# Autodesk Inventor assembly: X-axis Assembly
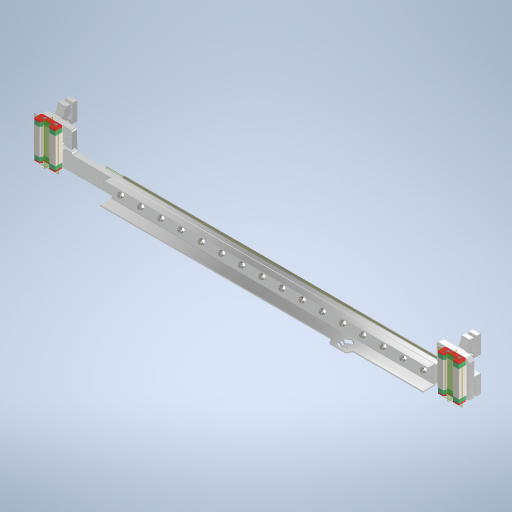
[picture p0: Inventor's stored thumbnail of the model, 512x512]
Saved by Autodesk Inventor 2024 (Build 280153000, 153)
## iProperties
Created: 2024-08-04
Part Number: X-axis Assembly
Document SubType Name: Assembly
Designer: Ishaan
Author: Ishaan
## Documents named in this file (9)
- E:\Projects\Axiom--IDEX-3D-Printer\CAD\12 - X-axis\X-axis Assembly.iam
- E:\Projects\Axiom--IDEX-3D-Printer\CAD\00 - COTS Components\MGN12H\MGN12H, LINEAR GUIDE BLOCK.ipt
- E:\Projects\Axiom--IDEX-3D-Printer\CAD\00 - COTS Components\MGNR12 400mm Rail\MGNR12R400HM.ipt
- E:\Projects\Axiom--IDEX-3D-Printer\CAD\12 - X-axis\Gantry Belt Clamp.ipt
- E:\Projects\Axiom--IDEX-3D-Printer\CAD\12 - X-axis\Gantry Stiffener.ipt
- E:\Projects\Axiom--IDEX-3D-Printer\CAD\00 - COTS Components\Hardware\SHCSM3x8.ipt
- E:\Projects\Axiom--IDEX-3D-Printer\CAD\00 - COTS Components\Hardware\SHCSM3x16.ipt
- E:\Projects\Axiom--IDEX-3D-Printer\CAD\00 - COTS Components\Hardware\M3 LOCKNUT.ipt
- E:\Projects\Axiom--IDEX-3D-Printer\CAD\12 - X-axis\R3 Gantry Bar.ipt
## Components (51 placed, 8 different names)
1. MGN12H, LINEAR GUIDE BLOCK:1
2. MGN12H, LINEAR GUIDE BLOCK:2
3. MGNR12R400HM:1 — Insert:121
4. R3 Gantry Bar:1
5. Gantry Belt Clamp:1 — Insert:119, Insert:120
6. Gantry Belt Clamp:2 — Insert:117, Insert:118
7. Gantry Stiffener:1 — Insert:122
8. SHCSM3x8:1
9. SHCSM3x8:2
10. SHCSM3x8:3
11. SHCSM3x8:4
12. SHCSM3x8:5
13. SHCSM3x8:6
14. SHCSM3x8:7
15. SHCSM3x8:8
16. SHCSM3x16:1 — Insert:117
17. SHCSM3x16:2 — Insert:118
18. SHCSM3x16:3 — Insert:119
19. SHCSM3x16:4 — Insert:120
20. SHCSM3x16:5 — Insert:121
21. SHCSM3x16:6
22. SHCSM3x16:7
23. SHCSM3x16:8
24. SHCSM3x16:9
25. SHCSM3x16:10
26. SHCSM3x16:11
27. SHCSM3x16:12
28. SHCSM3x16:13
29. SHCSM3x16:14
30. SHCSM3x16:15
31. SHCSM3x16:16
32. SHCSM3x16:17
33. SHCSM3x16:18
34. SHCSM3x16:19
35. SHCSM3x16:20
36. M3 LOCKNUT:1 — Insert:122
37. M3 LOCKNUT:2
38. M3 LOCKNUT:3
39. M3 LOCKNUT:4
40. M3 LOCKNUT:5
41. M3 LOCKNUT:6
42. M3 LOCKNUT:7
43. M3 LOCKNUT:8
44. M3 LOCKNUT:9
45. M3 LOCKNUT:10
46. M3 LOCKNUT:11
47. M3 LOCKNUT:12
48. M3 LOCKNUT:13
49. M3 LOCKNUT:14
50. M3 LOCKNUT:15
51. M3 LOCKNUT:16
## Component patterns: (16 elements, first: SHCSM3x16:5), (16 elements, first: M3 LOCKNUT:1)
## Relationships (59: Insert 59)
- [Insert]: MGN12H, LINEAR GUIDE BLOCK:1 ↔ R3 Gantry Bar:1
- [Insert]: MGN12H, LINEAR GUIDE BLOCK:1 ↔ R3 Gantry Bar:1
- [Insert]: MGN12H, LINEAR GUIDE BLOCK:1 ↔ R3 Gantry Bar:1
- [Insert]: MGN12H, LINEAR GUIDE BLOCK:1 ↔ R3 Gantry Bar:1
- [Insert]: MGN12H, LINEAR GUIDE BLOCK:2 ↔ R3 Gantry Bar:1
- [Insert]: MGN12H, LINEAR GUIDE BLOCK:2 ↔ R3 Gantry Bar:1
- [Insert]: MGN12H, LINEAR GUIDE BLOCK:2 ↔ R3 Gantry Bar:1
- [Insert]: MGN12H, LINEAR GUIDE BLOCK:2 ↔ R3 Gantry Bar:1
- [Insert]: MGNR12R400HM:1 ↔ R3 Gantry Bar:1
- [Insert]: MGNR12R400HM:1 ↔ R3 Gantry Bar:1
- [Insert]: MGNR12R400HM:1 ↔ R3 Gantry Bar:1
- [Insert]: MGNR12R400HM:1 ↔ R3 Gantry Bar:1
- [Insert]: MGNR12R400HM:1 ↔ R3 Gantry Bar:1
- [Insert]: MGNR12R400HM:1 ↔ R3 Gantry Bar:1
- [Insert]: MGNR12R400HM:1 ↔ R3 Gantry Bar:1
- [Insert]: MGNR12R400HM:1 ↔ R3 Gantry Bar:1
- [Insert]: MGNR12R400HM:1 ↔ R3 Gantry Bar:1
- [Insert]: MGNR12R400HM:1 ↔ R3 Gantry Bar:1
- [Insert]: MGNR12R400HM:1 ↔ R3 Gantry Bar:1
- [Insert]: MGNR12R400HM:1 ↔ R3 Gantry Bar:1
- [Insert]: MGNR12R400HM:1 ↔ R3 Gantry Bar:1
- [Insert]: MGNR12R400HM:1 ↔ R3 Gantry Bar:1
- [Insert]: MGNR12R400HM:1 ↔ R3 Gantry Bar:1
- [Insert]: MGNR12R400HM:1 ↔ R3 Gantry Bar:1
- [Insert]: MGNR12R400HM:1 ↔ R3 Gantry Bar:1
- [Insert] (0.1 mm): R3 Gantry Bar:1 ↔ Gantry Belt Clamp:2
- [Insert] (0.1 mm): R3 Gantry Bar:1 ↔ Gantry Belt Clamp:2
- [Insert] (0.1 mm): R3 Gantry Bar:1 ↔ Gantry Belt Clamp:1
- [Insert] (0.1 mm): R3 Gantry Bar:1 ↔ Gantry Belt Clamp:1
- [Insert]: R3 Gantry Bar:1 ↔ Gantry Stiffener:1
- [Insert]: R3 Gantry Bar:1 ↔ Gantry Stiffener:1
- [Insert]: R3 Gantry Bar:1 ↔ Gantry Stiffener:1
- [Insert]: R3 Gantry Bar:1 ↔ Gantry Stiffener:1
- [Insert]: R3 Gantry Bar:1 ↔ Gantry Stiffener:1
- [Insert]: R3 Gantry Bar:1 ↔ Gantry Stiffener:1
- [Insert]: R3 Gantry Bar:1 ↔ Gantry Stiffener:1
- [Insert]: R3 Gantry Bar:1 ↔ Gantry Stiffener:1
- [Insert]: R3 Gantry Bar:1 ↔ Gantry Stiffener:1
- [Insert]: R3 Gantry Bar:1 ↔ Gantry Stiffener:1
- [Insert]: R3 Gantry Bar:1 ↔ Gantry Stiffener:1
- [Insert]: R3 Gantry Bar:1 ↔ Gantry Stiffener:1
- [Insert]: R3 Gantry Bar:1 ↔ Gantry Stiffener:1
- [Insert]: R3 Gantry Bar:1 ↔ Gantry Stiffener:1
- [Insert]: R3 Gantry Bar:1 ↔ Gantry Stiffener:1
- [Insert]: R3 Gantry Bar:1 ↔ Gantry Stiffener:1
- [Insert]: R3 Gantry Bar:1 ↔ SHCSM3x8:8
- [Insert]: R3 Gantry Bar:1 ↔ SHCSM3x8:7
- [Insert]: R3 Gantry Bar:1 ↔ SHCSM3x8:5
- [Insert]: R3 Gantry Bar:1 ↔ SHCSM3x8:6
- [Insert]: R3 Gantry Bar:1 ↔ SHCSM3x8:4
- [Insert]: R3 Gantry Bar:1 ↔ SHCSM3x8:3
- [Insert]: R3 Gantry Bar:1 ↔ SHCSM3x8:1
- [Insert]: R3 Gantry Bar:1 ↔ SHCSM3x8:2
- Insert:117: Gantry Belt Clamp:2 ↔ SHCSM3x16:1
- Insert:118: Gantry Belt Clamp:2 ↔ SHCSM3x16:2
- Insert:119: Gantry Belt Clamp:1 ↔ SHCSM3x16:3
- Insert:120: Gantry Belt Clamp:1 ↔ SHCSM3x16:4
- Insert:121: MGNR12R400HM:1 ↔ SHCSM3x16:5
- Insert:122: Gantry Stiffener:1 ↔ M3 LOCKNUT:1
